# Autodesk Inventor assembly: GE-13020
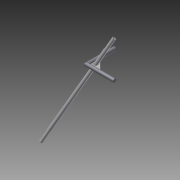
[picture p0: Inventor's stored thumbnail of the model, 180x180]
Saved by Autodesk Inventor 2013 (Build 170138000, 138)
## iProperties
Created: 2013-01-06
Part Number: GE-13020
Document SubType Name: Assembly
Designer: Phillip
_SolveAssemblyDoc: Frame Generator Solve Assembly
_Version: 15.0.0
Author: Phillip
## Documents named in this file (6)
- C:\Users\Moses\Documents\Inventor\2013 Team 3061 Robot\FIRST Arena 2013\Pyramid\GE-13020.iam
- C:\Users\Moses\Documents\Inventor\2013 Team 3061 Robot\FIRST Arena 2013\Pyramid\GE-13020Frame.ipt
- C:\Users\Moses\Documents\Inventor\2013 Team 3061 Robot\FIRST Arena 2013\Pyramid\GE-13020\Frame\Frame0001.iam
- C:\Users\Moses\Documents\Inventor\2013 Team 3061 Robot\FIRST Arena 2013\Pyramid\GE-13020-02.ipt
- C:\Users\Moses\Documents\Inventor\2013 Team 3061 Robot\FIRST Arena 2013\Pyramid\GE-13020-03.ipt
- C:\Users\Moses\Documents\Inventor\2013 Team 3061 Robot\FIRST Arena 2013\Pyramid\GE-13020-05.ipt
## Components (6 placed, 5 different names)
1. GE-13020Frame:1
2. Frame0001:1 [sub-assembly] — Mate:1, Tangent:1, Tangent:2
3. GE-13020-02:1 — Mate:1, Tangent:1, Tangent:2, Mate:2, Mate:3, Mate:4, Mate:5, Mate:6, Mate:7, Angle:1, Mate:10, Angle:2, Mate:16, Mate:17, Mate:18, Angle:5, Mate:26
4. GE-13020-03:1 — Mate:21, Mate:22, Mate:23, Flush:1, Flush:2
5. GE-13020-05:1 — Mate:22, Flush:1, Mate:24
6. GE-13020-05:2 — Mate:23, Flush:2
## Relationships (35: Mate 26, Angle 5, Tangent 2, Flush 2)
- Mate:1: Frame0001:1 ↔ GE-13020-02:1
- Tangent:1: Frame0001:1 ↔ GE-13020-02:1
- Tangent:2: Frame0001:1 ↔ GE-13020-02:1
- Mate:2: GE-13020-02:1
- Mate:3: GE-13020-02:1
- Mate:4: GE-13020-02:1
- Mate:5: GE-13020-02:1
- Mate:6: GE-13020-02:1
- Mate:7: GE-13020-02:1
- Angle:1 (0 deg): GE-13020-02:1
- Mate:8
- Mate:9
- Mate:10: GE-13020-02:1
- Mate:11
- Angle:2 (0 deg): GE-13020-02:1
- Mate:12
- Angle:3 (60 deg)
- Mate:13
- Angle:4 (90 deg)
- Mate:14
- Mate:15
- Mate:16: GE-13020-02:1
- Mate:17: GE-13020-02:1
- Mate:18: GE-13020-02:1
- Mate:19
- Mate:20
- Mate:21: GE-13020-03:1
- Mate:22: GE-13020-03:1 ↔ GE-13020-05:1
- Mate:23: GE-13020-03:1 ↔ GE-13020-05:2
- Flush:1 (-127 mm): GE-13020-03:1 ↔ GE-13020-05:1
- Flush:2 (127 mm): GE-13020-03:1 ↔ GE-13020-05:2
- Mate:24: GE-13020-05:1
- Mate:25
- Angle:5 (90 deg): GE-13020-02:1
- Mate:26: GE-13020-02:1
